# Autodesk Inventor assembly: INNER TORSO
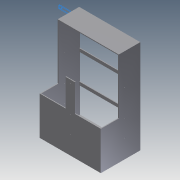
[picture p0: Inventor's stored thumbnail of the model, 180x180]
Saved by Autodesk Inventor 2011 (Build 150239000, 239)
## iProperties
Created: 2011-09-03
Part Number: INNER TORSO
Document SubType Name: Assembly
Designer: Matthew
Author: Matthew
## Documents named in this file (6)
- C:\Users\Matthew\Documents\matthew_autocad\prlite\inner torso\INNER TORSO.iam
- C:\Users\Matthew\Documents\matthew_autocad\prlite\inner torso\it side.ipt
- C:\Users\Matthew\Documents\matthew_autocad\prlite\inner torso\it front.ipt
- C:\Users\Matthew\Documents\matthew_autocad\prlite\inner torso\it top.ipt
- C:\Users\Matthew\Documents\matthew_autocad\prlite\inner torso\it bottom.ipt
- C:\Users\Matthew\Documents\matthew_autocad\prlite\inner torso\it (tech) support.ipt
## Components (8 placed, 5 different names)
1. it side:1 — Flush:5, Mate:7, Flush:18, Flush:19, Mate:18, Flush:26, Flush:28, Mate:20, Flush:29
2. it front:1 — Flush:5, Mate:7, Mate:11, Flush:17, Flush:19, Flush:23
3. it top:1 — Flush:24, Flush:25, Flush:26, Mate:22, Mate:24
4. it bottom:1 — Mate:11, Flush:17, Flush:18, Mate:15, Mate:18
5. it side:2 — Flush:23, Mate:15, Flush:24, Flush:25, Flush:27, Mate:21, Flush:30, Flush:31, Mate:23, Mate:24
6. it (tech) support:1 — Flush:30, Flush:31, Mate:23
7. it (tech) support:2 — Mate:21, Mate:22, Flush:29
8. it (tech) support:3 — Flush:27, Flush:28, Mate:20
## Relationships (22: Flush 13, Mate 9)
- Flush:5: it side:1 ↔ it front:1
- Mate:7: it side:1 ↔ it front:1
- Mate:11: it front:1 ↔ it bottom:1
- Flush:17: it front:1 ↔ it bottom:1
- Flush:18: it side:1 ↔ it bottom:1
- Flush:19: it side:1 ↔ it front:1
- Flush:23: it front:1 ↔ it side:2
- Mate:15: it bottom:1 ↔ it side:2
- Mate:18: it side:1 ↔ it bottom:1
- Flush:24: it top:1 ↔ it side:2
- Flush:25: it top:1 ↔ it side:2
- Flush:26: it side:1 ↔ it top:1
- Flush:27: it side:2 ↔ it (tech) support:3
- Flush:28: it side:1 ↔ it (tech) support:3
- Mate:20: it side:1 ↔ it (tech) support:3
- Mate:21: it side:2 ↔ it (tech) support:2
- Mate:22: it top:1 ↔ it (tech) support:2
- Flush:29: it side:1 ↔ it (tech) support:2
- Flush:30: it side:2 ↔ it (tech) support:1
- Flush:31: it side:2 ↔ it (tech) support:1
- Mate:23: it side:2 ↔ it (tech) support:1
- Mate:24: it top:1 ↔ it side:2
